# Autodesk Inventor assembly: Test stand v1.2
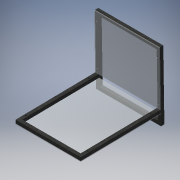
[picture p0: Inventor's stored thumbnail of the model, 180x180]
Saved by Autodesk Inventor 2019 (Build 230136000, 136)
## iProperties
Created: 2021-03-22
Part Number: Test stand v1.2
Document SubType Name: Assembly
Designer: User
Author: User
## Documents named in this file (6)
- C:\Users\User\Desktop\Test Stand\Test stand v1.2.iam
- C:\Users\User\Desktop\Test Stand\Base395.ipt
- C:\Users\User\Desktop\Test Stand\Base 335.ipt
- C:\Users\User\Desktop\Test Stand\height 460.ipt
- C:\Users\User\Desktop\Test Stand\perspex height.ipt
- C:\Users\User\Desktop\Test Stand\Perspex base.ipt
## Components (9 placed, 5 different names)
1. Base395:1 — Mate:1, Mate:2, Mate:3, Mate:7, Mate:8, Mate:9, Mate:12, Mate:13, Mate:22, Mate:23
2. Base395:3 — Mate:4, Mate:5, Mate:6, Mate:10, Mate:16
3. Base 335:1 — Mate:1, Mate:2, Mate:3, Mate:4, Mate:5, Mate:6, Mate:21, Mate:24
4. Base 335:2 — Mate:7, Mate:8, Mate:9
5. height 460:1 — Mate:12, Mate:13, Mate:18, Mate:19, Mate:25
6. height 460:2 — Mate:10, Mate:14, Mate:15, Mate:16, Mate:17
7. Base 335:3 — Mate:14, Mate:15, Mate:17, Mate:18, Mate:20
8. perspex height:1 — Mate:19, Mate:20
9. Perspex base:1 — Mate:21, Mate:22, Mate:23, Mate:24, Mate:25
## Relationships (24: Mate 24)
- Mate:1: Base395:1 ↔ Base 335:1
- Mate:2: Base395:1 ↔ Base 335:1
- Mate:3: Base395:1 ↔ Base 335:1
- Mate:4: Base395:3 ↔ Base 335:1
- Mate:5: Base395:3 ↔ Base 335:1
- Mate:6: Base395:3 ↔ Base 335:1
- Mate:7: Base395:1 ↔ Base 335:2
- Mate:8: Base395:1 ↔ Base 335:2
- Mate:9: Base395:1 ↔ Base 335:2
- Mate:10: Base395:3 ↔ height 460:2
- Mate:12: Base395:1 ↔ height 460:1
- Mate:13: Base395:1 ↔ height 460:1
- Mate:14: height 460:2 ↔ Base 335:3
- Mate:15: height 460:2 ↔ Base 335:3
- Mate:16: Base395:3 ↔ height 460:2
- Mate:17: height 460:2 ↔ Base 335:3
- Mate:18: height 460:1 ↔ Base 335:3
- Mate:19: height 460:1 ↔ perspex height:1
- Mate:20: Base 335:3 ↔ perspex height:1
- Mate:21: Base 335:1 ↔ Perspex base:1
- Mate:22: Base395:1 ↔ Perspex base:1
- Mate:23: Base395:1 ↔ Perspex base:1
- Mate:24: Base 335:1 ↔ Perspex base:1
- Mate:25: height 460:1 ↔ Perspex base:1
